# Autodesk Inventor assembly: IMS-10-000
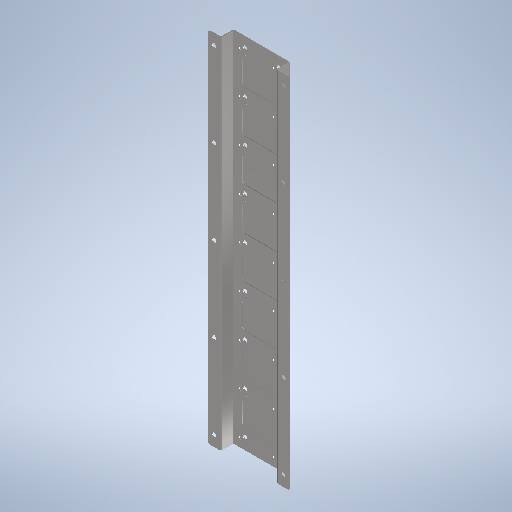
[picture p0: Inventor's stored thumbnail of the model, 512x512]
Saved by Autodesk Inventor 2025.2 (Build 292293000, 293)
## iProperties
Created: 2020-10-06
Part Number: IMS-10-000
Document SubType Name: Assembly
Designer: mahra
Mass: 4944.25 g
Surface Area: 5566.25 cm^2
Volume: 642.136 cm^3
Density: 7.69969 g/cm^3
Author: mahra
## Documents named in this file (3)
- C:\Users\Caspe\Documents\Semester 8\Project\Anomaly_Detection\Mechanical_Project\Inventor_project\IMS-10-000.iam
- C:\Users\Caspe\Documents\Semester 8\Project\Anomaly_Detection\Mechanical_Project\Inventor_project\IMS-10-001.ipt
- C:\Users\Caspe\Documents\Semester 8\Project\Anomaly_Detection\Mechanical_Project\Inventor_project\IMS-10-002.ipt
## Components (2 placed, 2 different names)
1. IMS-10-001:1 — Mate:1, Flush:1, Flush:2
2. IMS-10-002:1 — Mate:1, Flush:1, Flush:2
## Relationships (3: Flush 2, Mate 1)
- Mate:1: IMS-10-001:1 ↔ IMS-10-002:1
- Flush:1 (7.5 mm): IMS-10-001:1 ↔ IMS-10-002:1
- Flush:2 (5 mm): IMS-10-001:1 ↔ IMS-10-002:1
